# Autodesk Inventor assembly: 42146-35
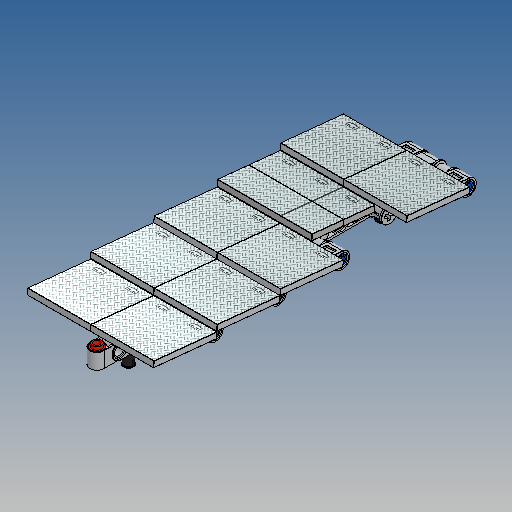
[picture p0: Inventor's stored thumbnail of the model, 512x512]
Saved by Autodesk Inventor 2025 (Build 290162010, 162A)
## iProperties
Created: 2024-12-07
Part Number: 42146-35
Material: Generisch
Document SubType Name: Assembly
Designer: hp.muther
Author: hp.muther
## Documents named in this file (10)
- D:\Inventor\Projekte\Muther\LEGO Technic\LEGO Technik - Raupenkran LR 13000 (42146)\42146-35.iam
- D:\Inventor\Projekte\Muther\LEGO Technic\LEGO Pieces\Lochbalken\73507-LtBluishGray.ipt
- D:\Inventor\Projekte\Muther\LEGO Technic\LEGO Pieces\Pin's\2780-Black.ipt
- D:\Inventor\Projekte\Muther\LEGO Technic\LEGO Pieces\Pin's\43093-Blue.ipt
- D:\Inventor\Projekte\Muther\LEGO Technic\LEGO Pieces\Pin's\32054-LtBluishGray.ipt
- D:\Inventor\Projekte\Muther\LEGO Technic\LEGO Pieces\Platten, Kacheln\43045-LtBluishGray.ipt
- D:\Inventor\Projekte\Muther\LEGO Technic\LEGO Pieces\Pin's\4274-Red.ipt
- D:\Inventor\Projekte\Muther\LEGO Technic\LEGO Technik - Raupenkran LR 13000 (42146)\42146_1751_1.ipt
- D:\Inventor\Projekte\Muther\LEGO Technic\LEGO Technik - Raupenkran LR 13000 (42146)\42146_69729_2.ipt
- D:\Inventor\Projekte\Muther\LEGO Technic\LEGO Technik - Raupenkran LR 13000 (42146)\42146_69729_3.ipt
## Components (37 placed, 9 different names)
1. 73507-LtBluishGray:1 — Einfügen:1, Einfügen:2, Einfügen:3, Einfügen:7, Fluchtend:2, Fluchtend:3, Passend:1, Einfügen:13, Einfügen:17
2. 2780-Black:1 — Einfügen:3
3. 2780-Black:2 — Einfügen:1
4. 2780-Black:3 — Einfügen:2
5. 43093-Blue:1 — Einfügen:4, Einfügen:5
6. 32054-LtBluishGray:1 — Einfügen:4, Einfügen:6, Einfügen:7
7. 43045-LtBluishGray:1 — Einfügen:6, Fluchtend:1, Winkel:2, Passend:2, Passend:3, Passend:5, Fluchtend:5
8. 43045-LtBluishGray:2 — Einfügen:5, Fluchtend:1, Passend:6
9. 73507-LtBluishGray:2 — Einfügen:8, Einfügen:9, Einfügen:10, Fluchtend:2, Fluchtend:3, Passend:1, Einfügen:11, Einfügen:24, Einfügen:25
10. 2780-Black:4 — Einfügen:9
11. 2780-Black:5 — Einfügen:8
12. 2780-Black:6 — Einfügen:10
13. 4274-Red:1 — Einfügen:11
14. 32054-LtBluishGray:2 — Einfügen:12, Einfügen:13
15. 43045-LtBluishGray:3 — Einfügen:12, Winkel:2, Passend:2, Passend:8, Passend:9, Passend:11, Passend:12, Passend:17
16. 42146_1751_1:1 — Passend:6, Passend:7, Fluchtend:6
17. 42146_1751_1:2 — Passend:3, Passend:5, Fluchtend:5, Passend:7, Fluchtend:6
18. 42146_69729_2:1 — Passend:9, Passend:10, Passend:11, Fluchtend:7
19. 42146_69729_3:1 — Passend:8, Passend:10, Passend:12, Fluchtend:7
20. 43093-Blue:2
21. 32054-LtBluishGray:3 — Einfügen:17
22. 43045-LtBluishGray:4 — Passend:17
23. 43045-LtBluishGray:5
24. 42146_1751_1:3
25. 42146_1751_1:4
26. 43093-Blue:3
27. 32054-LtBluishGray:4 — Einfügen:24
28. 43045-LtBluishGray:6 — Passend:26
29. 43045-LtBluishGray:7
30. 42146_1751_1:5
31. 42146_1751_1:6
32. 43093-Blue:4
33. 32054-LtBluishGray:5 — Einfügen:25
34. 43045-LtBluishGray:8 — Passend:26
35. 43045-LtBluishGray:9
36. 42146_1751_1:7
37. 42146_1751_1:8
## Relationships (66: Insert 25, Mate 25, Flush 15, Angle 1)
- Einfügen:1 [Insert]: 73507-LtBluishGray:1 ↔ 2780-Black:2
- Einfügen:2 [Insert]: 73507-LtBluishGray:1 ↔ 2780-Black:3
- Einfügen:3 [Insert]: 73507-LtBluishGray:1 ↔ 2780-Black:1
- Einfügen:4 [Insert]: 43093-Blue:1 ↔ 32054-LtBluishGray:1
- Einfügen:5 [Insert]: 43093-Blue:1 ↔ 43045-LtBluishGray:2
- Einfügen:6 [Insert] (8 mm): 32054-LtBluishGray:1 ↔ 43045-LtBluishGray:1
- Fluchtend:1 [Flush]: 43045-LtBluishGray:1 ↔ 43045-LtBluishGray:2
- Einfügen:7 [Insert]: 73507-LtBluishGray:1 ↔ 32054-LtBluishGray:1
- Passend:2 [Mate]: 43045-LtBluishGray:1 ↔ 43045-LtBluishGray:3
- Einfügen:8 [Insert]: 73507-LtBluishGray:2 ↔ 2780-Black:5
- Einfügen:9 [Insert]: 73507-LtBluishGray:2 ↔ 2780-Black:4
- Einfügen:10 [Insert]: 73507-LtBluishGray:2 ↔ 2780-Black:6
- Fluchtend:2 [Flush]: 73507-LtBluishGray:1 ↔ 73507-LtBluishGray:2
- Fluchtend:3 [Flush]: 73507-LtBluishGray:1 ↔ 73507-LtBluishGray:2
- Passend:1 [Mate] (-56 mm): 73507-LtBluishGray:1 ↔ 73507-LtBluishGray:2
- Einfügen:11 [Insert]: 73507-LtBluishGray:2 ↔ 4274-Red:1
- Einfügen:12 [Insert] (8 mm): 32054-LtBluishGray:2 ↔ 43045-LtBluishGray:3
- Einfügen:13 [Insert]: 73507-LtBluishGray:1 ↔ 32054-LtBluishGray:2
- Winkel:2 [Angle] (0 deg): 43045-LtBluishGray:1 ↔ 43045-LtBluishGray:3
- Passend:3 [Mate]: 43045-LtBluishGray:1 ↔ 42146_1751_1:2
- Passend:5 [Mate] (8 mm): 43045-LtBluishGray:1 ↔ 42146_1751_1:2
- Fluchtend:5 [Flush]: 43045-LtBluishGray:1 ↔ 42146_1751_1:2
- Passend:6 [Mate]: 43045-LtBluishGray:2 ↔ 42146_1751_1:1
- Passend:7 [Mate]: 42146_1751_1:1 ↔ 42146_1751_1:2
- Fluchtend:6 [Flush]: 42146_1751_1:1 ↔ 42146_1751_1:2
- Passend:8 [Mate]: 43045-LtBluishGray:3 ↔ 42146_69729_3:1
- Passend:9 [Mate]: 43045-LtBluishGray:3 ↔ 42146_69729_2:1
- Passend:10 [Mate]: 42146_69729_2:1 ↔ 42146_69729_3:1
- Passend:11 [Mate] (8 mm): 43045-LtBluishGray:3 ↔ 42146_69729_2:1
- Passend:12 [Mate] (-32 mm): 43045-LtBluishGray:3 ↔ 42146_69729_3:1
- Fluchtend:7 [Flush]: 42146_69729_2:1 ↔ 42146_69729_3:1
- [Insert]: 43093-Blue:2 ↔ 32054-LtBluishGray:3
- [Insert]: 43093-Blue:2 ↔ 43045-LtBluishGray:5
- [Insert] (8 mm): 32054-LtBluishGray:3 ↔ 43045-LtBluishGray:4
- [Flush]: 43045-LtBluishGray:4 ↔ 43045-LtBluishGray:5
- [Mate]: 43045-LtBluishGray:4 ↔ 42146_1751_1:4
- [Mate] (8 mm): 43045-LtBluishGray:4 ↔ 42146_1751_1:4
- [Flush]: 43045-LtBluishGray:4 ↔ 42146_1751_1:4
- [Mate]: 43045-LtBluishGray:5 ↔ 42146_1751_1:3
- [Mate]: 42146_1751_1:3 ↔ 42146_1751_1:4
- [Flush]: 42146_1751_1:3 ↔ 42146_1751_1:4
- Einfügen:17 [Insert]: 73507-LtBluishGray:1 ↔ 32054-LtBluishGray:3
- Passend:17 [Mate]: 43045-LtBluishGray:3 ↔ 43045-LtBluishGray:4
- [Insert]: 43093-Blue:3 ↔ 32054-LtBluishGray:4
- [Insert]: 43093-Blue:3 ↔ 43045-LtBluishGray:7
- [Insert] (8 mm): 32054-LtBluishGray:4 ↔ 43045-LtBluishGray:6
- [Flush]: 43045-LtBluishGray:6 ↔ 43045-LtBluishGray:7
- [Mate]: 43045-LtBluishGray:6 ↔ 42146_1751_1:6
- [Mate] (8 mm): 43045-LtBluishGray:6 ↔ 42146_1751_1:6
- [Flush]: 43045-LtBluishGray:6 ↔ 42146_1751_1:6
- [Mate]: 43045-LtBluishGray:7 ↔ 42146_1751_1:5
- [Mate]: 42146_1751_1:5 ↔ 42146_1751_1:6
- [Flush]: 42146_1751_1:5 ↔ 42146_1751_1:6
- [Insert]: 43093-Blue:4 ↔ 32054-LtBluishGray:5
- [Insert]: 43093-Blue:4 ↔ 43045-LtBluishGray:9
- [Insert] (8 mm): 32054-LtBluishGray:5 ↔ 43045-LtBluishGray:8
- [Flush]: 43045-LtBluishGray:8 ↔ 43045-LtBluishGray:9
- [Mate]: 43045-LtBluishGray:8 ↔ 42146_1751_1:8
- [Mate] (8 mm): 43045-LtBluishGray:8 ↔ 42146_1751_1:8
- [Flush]: 43045-LtBluishGray:8 ↔ 42146_1751_1:8
- [Mate]: 43045-LtBluishGray:9 ↔ 42146_1751_1:7
- [Mate]: 42146_1751_1:7 ↔ 42146_1751_1:8
- [Flush]: 42146_1751_1:7 ↔ 42146_1751_1:8
- Einfügen:24 [Insert]: 73507-LtBluishGray:2 ↔ 32054-LtBluishGray:4
- Einfügen:25 [Insert]: 73507-LtBluishGray:2 ↔ 32054-LtBluishGray:5
- Passend:26 [Mate]: 43045-LtBluishGray:6 ↔ 43045-LtBluishGray:8
## Named parameters: d9_d0 = 0 mm, d10_d2 = 0 mm, d16_d5 = 8 mm, d32_d22 = 0 mm, d33_d23 = 0 mm, d34_d24 = 0 mm, d35_d25 = 0 mm, d36_d4 = 0 mm, d37_d5 = 8 mm, d38_d6 = 0 mm, d39_d20 = 0 mm, d40_d21 = 8 mm, d41_d3 = 0 mm, d44_d22 = 0 mm, d45_d23 = 0 mm, d46_d24 = 0 mm, d47_d25 = 0 mm, d48_d4 = 0 mm, d49_d5 = 8 mm, d50_d6 = 0 mm, d51_d20 = 0 mm, d52_d21 = 8 mm, d53_d3 = 0 mm, d54_d22 = 0 mm, d55_d23 = 0 mm, d56_d24 = 0 mm, d57_d25 = 0 mm, d58_d4 = 0 mm, d59_d5 = 8 mm, d60_d6 = 0 mm, d61_d20 = 0 mm, d62_d21 = 8 mm, d63_d3 = 0 mm
